# Autodesk Inventor assembly: tank_sensorssupport_assembly
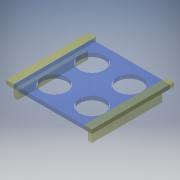
[picture p0: Inventor's stored thumbnail of the model, 180x180]
Saved by Autodesk Inventor 2018.1 (Build 221171000, 171)
## iProperties
Created: 2017-08-15
Part Number: tank_sensorssupport_assembly
Document SubType Name: Assembly
Designer: Tom
Mass: 56.6573 g
Surface Area: 267.278 cm^2
Volume: 40.4695 cm^3
Density: 1.4 g/cm^3
Author: Tom
## Documents named in this file (5)
- \\Mac\Dropbox\2015-2016\Bachelorproef\Inventor\Etstank_v2\tank_sensorssupport_assembly.iam
- \\Mac\Dropbox\2015-2016\Bachelorproef\Inventor\Etstank_v2\tank_sensorssupport.ipt
- \\Mac\Dropbox\2015-2016\Bachelorproef\Inventor\Etstank_v2\tank_bracket_short_top.ipt
- \\Mac\Dropbox\2015-2016\Bachelorproef\Inventor\Etstank_v2\tank_bracket_short_bottom.ipt
- \\Mac\Dropbox\2015-2016\Bachelorproef\Inventor\Etstank_v2\par.xls
## Components (5 placed, 3 different names)
1. tank_sensorssupport:1 — Mate:1, Mate:2, Flush:3, Flush:4, Flush:5, Flush:6, Flush:9, Flush:10, Mate:3, Flush:11, Flush:12, Flush:13, Mate:4, Flush:14
2. tank_bracket_short_top:1 — Mate:1, Flush:4, Flush:6
3. tank_bracket_short_top:2 — Mate:2, Flush:3, Flush:5
4. tank_bracket_short_bottom:1 — Flush:9, Mate:3, Flush:11, Flush:12
5. tank_bracket_short_bottom:2 — Flush:10, Flush:13, Mate:4, Flush:14
## Relationships (14: Flush 10, Mate 4)
- Mate:1: tank_sensorssupport:1 ↔ tank_bracket_short_top:1
- Mate:2: tank_sensorssupport:1 ↔ tank_bracket_short_top:2
- Flush:3 (5 mm): tank_sensorssupport:1 ↔ tank_bracket_short_top:2
- Flush:4 (-5 mm): tank_sensorssupport:1 ↔ tank_bracket_short_top:1
- Flush:5: tank_sensorssupport:1 ↔ tank_bracket_short_top:2
- Flush:6: tank_sensorssupport:1 ↔ tank_bracket_short_top:1
- Flush:9: tank_sensorssupport:1 ↔ tank_bracket_short_bottom:1
- Flush:10: tank_sensorssupport:1 ↔ tank_bracket_short_bottom:2
- Mate:3: tank_sensorssupport:1 ↔ tank_bracket_short_bottom:1
- Flush:11: tank_sensorssupport:1 ↔ tank_bracket_short_bottom:1
- Flush:12: tank_sensorssupport:1 ↔ tank_bracket_short_bottom:1
- Flush:13: tank_sensorssupport:1 ↔ tank_bracket_short_bottom:2
- Mate:4: tank_sensorssupport:1 ↔ tank_bracket_short_bottom:2
- Flush:14: tank_sensorssupport:1 ↔ tank_bracket_short_bottom:2
## Named parameters: maxl = 400 mm, maxh = 400 mm, maxw = 350 mm, lcsd = 19.05 mm, lcdd = 100 mm, lcwd1 = 25 mm, lcwd2 = 34 mm, lcw = 20 mm, lch1 = 39 mm, lch2 = 40 mm, lcl = 150 mm, lcwd3 = 43 mm, dia1 = 6 mm, td = 18 mm, bhh = 6 mm, bhd = 10 mm, sw = 25 mm, sh = 31 mm, spacert = 2 mm, nutdist = 40 mm, platft = 20 mm, supt = 20 mm, pvct = 5 mm, tankw = 100 mm, tankh = 370 mm, tankl = 379 mm, dia2 = 20 mm, tankv = 1e+07 mm, actual_tankv = 1.4023e+07 mm, dia4 = 11 mm, dia3 = 8 mm, play = 9 mm, holeh = 26 mm, surroundh = 60 mm, slack = 0.5 mm, surroundt = 5 mm, play2 = 3 mm, extra_height = 100 mm, diaair = 32 mm, diaph = 32 mm, diawater = 25 mm, diacucl = 32 mm, diafloat = 50 mm, diahcl = 32 mm, diaoverflow = 25 mm, mindist = 80 mm, distfromedge = 10 mm, diasurroundhole = 42 mm, bracketw = 10 mm, bracketwbottom = 6 mm, sensorsupportl = 100 mm, diagrate = 12 mm, gratespacing = 12.02082 mm, bottomdist = 9.6355 mm, sidedist = 13.9375 mm, handlel = 120 mm, handlesupporth = 20 mm, handlew = 50 mm, nett = 1 mm, netholespacing = 2 mm, nethole = 16 mm, nettop = 7 mm, netside = 3.5 mm, nutholdert = 10 mm, diaetape = 32 mm
